# Autodesk Inventor assembly: Motor
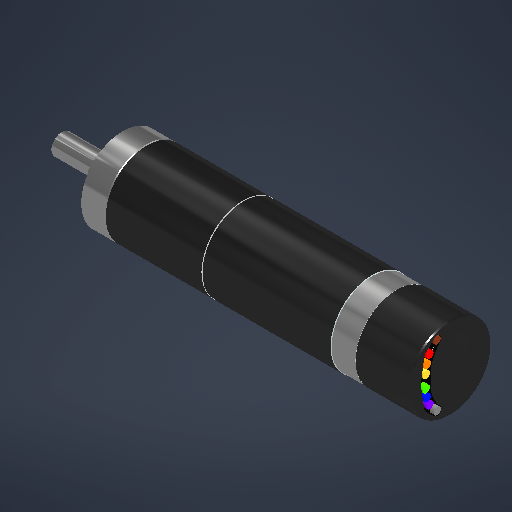
[picture p0: Inventor's stored thumbnail of the model, 512x512]
Saved by Autodesk Inventor 2026.1 (Build 301233020, 233B)
## iProperties
Created: 2024-10-01
Part Number: Motor
Document SubType Name: Assembly
Designer: theod
Author: theod
## Documents named in this file (3)
- C:\Users\Bahaa\Nextcloud2\CAD\25-26\Motoren\Motor.iam
- C:\Users\Bahaa\Nextcloud2\CAD\25-26\Motoren\400160_ec16_30w_a.ipt
- C:\Users\Bahaa\Nextcloud2\CAD\25-26\Motoren\407883_GP16C_0_3NM_2ST_KL.ipt
## Components (2 placed, 2 different names)
1. 400160_ec16_30w_a:1 — Mate:1, Mate:2, Mate:3
2. 407883_GP16C_0_3NM_2ST_KL:1 — Mate:1, Mate:2, Mate:3
## Relationships (3: Mate 3)
- Mate:1: 400160_ec16_30w_a:1 ↔ 407883_GP16C_0_3NM_2ST_KL:1
- Mate:2: 400160_ec16_30w_a:1 ↔ 407883_GP16C_0_3NM_2ST_KL:1
- Mate:3: 400160_ec16_30w_a:1 ↔ 407883_GP16C_0_3NM_2ST_KL:1
